# Autodesk Inventor assembly: PlanetaryGearConstr
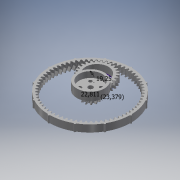
[picture p0: Inventor's stored thumbnail of the model, 180x180]
Saved by Autodesk Inventor 2018.3 (Build 223284000, 284)
## iProperties
Created: 2018-07-08
Part Number: PlanetaryGearConstr
Material: Generisch
Document SubType Name: Assembly
Designer: JochenAlt
Author: JochenAlt
## Documents named in this file (4)
- D:\Projects\FlowerPot\CAD\PlanetaryGear\PlanetaryGearConstr.iam
- D:\Projects\FlowerPot\CAD\PlanetaryGear\Konstruktions-Assistent\Stirnräder1.iam
- D:\Projects\FlowerPot\CAD\PlanetaryGear\Konstruktions-Assistent\Stirnräder3.iam
- D:\Projects\FlowerPot\CAD\PlanetaryGear\PlanetaryGearConstr\Konstruktions-Assistent\Stirnräder2.iam
## Components (3 placed, 1 different names)
1. Stirnräder:1 [sub-assembly] — Fluchtend:1, Fluchtend:2
2. Stirnräder:2 [sub-assembly] — Fluchtend:2, Passend:4
3. Stirnräder:3 [sub-assembly] — Fluchtend:1, Passend:2
## Relationships (4: Flush 2, Mate 2)
- Fluchtend:1 [Flush]: Stirnräder:1 ↔ Stirnräder:3
- Passend:2 [Mate]: Stirnräder:3
- Fluchtend:2 [Flush]: Stirnräder:1 ↔ Stirnräder:2
- Passend:4 [Mate] (18.538 mm): Stirnräder:2
